# Autodesk Inventor assembly: ElectricalAssembly
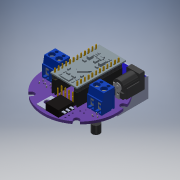
[picture p0: Inventor's stored thumbnail of the model, 180x180]
Saved by Autodesk Inventor 2018 (Build 220112000, 112)
## iProperties
Created: 2017-04-09
Part Number: ElectricalAssembly
Document SubType Name: Assembly
Designer: dkt01
Author: dkt01
## Documents named in this file (4)
- C:\Users\dktur\Dropbox\StackLightMonitor\CAD\ElectricalAssembly.iam
- C:\Users\dktur\Dropbox\StackLightMonitor\CAD\Shield.iam
- C:\Users\dktur\Dropbox\StackLightMonitor\CAD\ArduinoProMicro.iam
- C:\Users\dktur\Dropbox\StackLightMonitor\CAD\Ethernet.iam
## Components (3 placed, 3 different names)
1. Shield:1 [sub-assembly] — Mate:1, Flush:1, Flush:2, Mate:2, Tangent:1, Tangent:2, Tangent:3, Tangent:4, Mate:3, Mate:4
2. ArduinoProMicro:1 [sub-assembly] — Mate:1, Flush:1, Flush:2
3. Ethernet:1 [sub-assembly] — Mate:2, Tangent:1, Tangent:2, Tangent:3, Tangent:4
## Relationships (10: Mate 4, Tangent 4, Flush 2)
- Mate:1: Shield:1 ↔ ArduinoProMicro:1
- Flush:1: Shield:1 ↔ ArduinoProMicro:1
- Flush:2: Shield:1 ↔ ArduinoProMicro:1
- Mate:2: Shield:1 ↔ Ethernet:1
- Tangent:1: Shield:1 ↔ Ethernet:1
- Tangent:2: Shield:1 ↔ Ethernet:1
- Tangent:3: Shield:1 ↔ Ethernet:1
- Tangent:4: Shield:1 ↔ Ethernet:1
- Mate:3: Shield:1
- Mate:4: Shield:1
